# Autodesk Inventor assembly: s-assyypanel
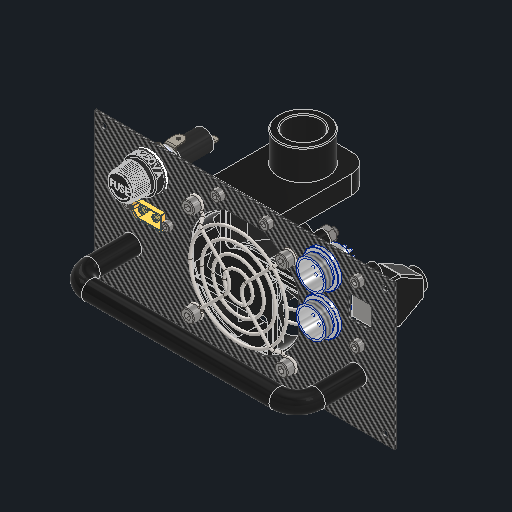
[picture p0: Inventor's stored thumbnail of the model, 512x512]
Saved by Autodesk Inventor 2022 (Build 260153000, 153)
## iProperties
Created: 2021-07-22
Part Number: s-assyypanel
Document SubType Name: Assembly
Designer: yuta0
Author: yuta0
## Documents named in this file (16)
- C:\Users\yuta0\Documents\GitHub\catchrobo_hardware\assy-scara\s-assyypanel.iam
- C:\Users\yuta0\Documents\GitHub\catchrobo_hardware\assy-scara\carbon_plate8.ipt
- C:\Users\yuta0\Documents\GitHub\catchrobo_hardware\assy-scara\Fan_Assembly.iam
- C:\Users\yuta0\Documents\GitHub\catchrobo_hardware\assy-scara\Fan protection grill 55023 - 60mm X 60mm.ipt
- C:\Users\yuta0\Documents\GitHub\catchrobo_hardware\assy-scara\SF372 10A 250VAC Fuse Holder.iam
- C:\Users\yuta0\Documents\GitHub\catchrobo_hardware\assy-scara\base11.ipt
- C:\Users\yuta0\Documents\GitHub\catchrobo_hardware\assy-scara\XT60E-M_V1.1.ipt
- C:\Users\yuta0\Documents\GitHub\catchrobo_hardware\assy-scara\UWANK10-120-27.ipt
- C:\Users\yuta0\Documents\GitHub\catchrobo_hardware\assy-scara\SB-305060.ipt
- C:\Users\yuta0\Documents\GitHub\catchrobo_hardware\assy-scara\CB3-5.ipt
- C:\Users\yuta0\Documents\GitHub\catchrobo_hardware\assy-scara\CB4-25.ipt
- C:\Users\yuta0\Documents\GitHub\catchrobo_hardware\assy-scara\LBNR4.ipt
- C:\Users\yuta0\Documents\GitHub\catchrobo_hardware\assy-scara\PLT-164-R-R.ipt
- C:\Users\yuta0\Documents\GitHub\catchrobo_hardware\assy-scara\USB2-MBMPAF-XXE.ipt
- C:\Users\yuta0\Documents\GitHub\catchrobo_hardware\assy-scara\CB2_5-6.ipt
- C:\Users\yuta0\Documents\GitHub\catchrobo_hardware\assy-scara\PLT-166-R-R.ipt
## Components (27 placed, 15 different names)
1. carbon_plate8:1 — メイト:10, メイト:12, メイト:13, メイト:14, メイト:15, 正接:1, メイト:21, メイト:22, 角度:2, メイト:27, メイト:28, メイト:30, メイト:31, メイト:32, メイト:33, メイト:34, メイト:35, メイト:40, メイト:41, メイト:42, メイト:43, メイト:44, メイト:46, メイト:47, メイト:48, メイト:49, メイト:50, メイト:51, メイト:54, メイト:55, メイト:56
2. PLT-164-R-R:1 — メイト:10, メイト:12, 角度:2
3. Fan_Assembly:1 [sub-assembly] — メイト:13, メイト:14, メイト:15, フラッシュ:1, メイト:16, メイト:25, メイト:26, 正接:2, メイト:29
4. Fan protection grill 55023 - 60mm X 60mm:1 — フラッシュ:1, メイト:16, 正接:1, 正接:3
5. SF372 10A 250VAC Fuse Holder:1 [sub-assembly] — メイト:21, メイト:22, 角度:1
6. Fan protection grill 55023 - 60mm X 60mm:2 — メイト:25, メイト:26, 正接:2, 正接:4
7. base11:1 — メイト:27, メイト:28, メイト:29, メイト:36, メイト:37, メイト:38, メイト:39
8. XT60E-M_V1.1:1 — メイト:30, メイト:31, メイト:32
9. UWANK10-120-27:1 — メイト:33, メイト:34, メイト:35
10. SB-305060:1 — メイト:36, メイト:39
11. SB-305060:2 — メイト:37, メイト:38
12. CB3-5:1 — メイト:42, メイト:43, メイト:53
13. CB3-5:2 — メイト:40, メイト:41, メイト:52
14. CB3-5:3 — メイト:46, メイト:47
15. CB3-5:4 — メイト:48, メイト:49
16. USB2-MBMPAF-XXE:1 — メイト:52, メイト:53, メイト:54
17. PLT-166-R-R:1 — メイト:55, メイト:56
18. CB4-25:1 — メイト:44, 正接:3, メイト:45
19. LBNR4:1 — メイト:45, 正接:4
20. CB4-25:2
21. LBNR4:2
22. CB4-25:3
23. LBNR4:3
24. CB4-25:4
25. LBNR4:4
26. CB2_5-6:1 — メイト:50, メイト:51
27. CB2_5-6:2
## Component patterns: (4 elements, first: CB4-25:1 + LBNR4:1), (2 elements, first: CB2_5-6:1)
## Relationships (47: Mate 40, Tangent 4, Angle 2, Flush 1)
- メイト:10 [Mate]: carbon_plate8:1 ↔ PLT-164-R-R:1
- メイト:12 [Mate]: carbon_plate8:1 ↔ PLT-164-R-R:1
- メイト:13 [Mate]: carbon_plate8:1 ↔ Fan_Assembly:1
- メイト:14 [Mate]: carbon_plate8:1 ↔ Fan_Assembly:1
- メイト:15 [Mate]: carbon_plate8:1 ↔ Fan_Assembly:1
- フラッシュ:1 [Flush]: Fan_Assembly:1 ↔ Fan protection grill 55023 - 60mm X 60mm:1
- メイト:16 [Mate]: Fan_Assembly:1 ↔ Fan protection grill 55023 - 60mm X 60mm:1
- 正接:1 [Tangent]: carbon_plate8:1 ↔ Fan protection grill 55023 - 60mm X 60mm:1
- メイト:21 [Mate]: carbon_plate8:1 ↔ SF372 10A 250VAC Fuse Holder:1
- メイト:22 [Mate]: carbon_plate8:1 ↔ SF372 10A 250VAC Fuse Holder:1
- 角度:1 [Angle] (0 deg): SF372 10A 250VAC Fuse Holder:1
- 角度:2 [Angle] (180 deg): carbon_plate8:1 ↔ PLT-164-R-R:1
- メイト:25 [Mate]: Fan_Assembly:1 ↔ Fan protection grill 55023 - 60mm X 60mm:2
- メイト:26 [Mate]: Fan_Assembly:1 ↔ Fan protection grill 55023 - 60mm X 60mm:2
- 正接:2 [Tangent]: Fan_Assembly:1 ↔ Fan protection grill 55023 - 60mm X 60mm:2
- メイト:27 [Mate]: carbon_plate8:1 ↔ base11:1
- メイト:28 [Mate]: carbon_plate8:1 ↔ base11:1
- メイト:29 [Mate]: Fan_Assembly:1 ↔ base11:1
- メイト:30 [Mate]: carbon_plate8:1 ↔ XT60E-M_V1.1:1
- メイト:31 [Mate]: carbon_plate8:1 ↔ XT60E-M_V1.1:1
- メイト:32 [Mate]: carbon_plate8:1 ↔ XT60E-M_V1.1:1
- メイト:33 [Mate]: carbon_plate8:1 ↔ UWANK10-120-27:1
- メイト:34 [Mate]: carbon_plate8:1 ↔ UWANK10-120-27:1
- メイト:35 [Mate]: carbon_plate8:1 ↔ UWANK10-120-27:1
- メイト:36 [Mate]: base11:1 ↔ SB-305060:1
- メイト:37 [Mate]: base11:1 ↔ SB-305060:2
- メイト:38 [Mate]: base11:1 ↔ SB-305060:2
- メイト:39 [Mate]: base11:1 ↔ SB-305060:1
- メイト:40 [Mate]: carbon_plate8:1 ↔ CB3-5:2
- メイト:41 [Mate]: carbon_plate8:1 ↔ CB3-5:2
- メイト:42 [Mate]: carbon_plate8:1 ↔ CB3-5:1
- メイト:43 [Mate]: carbon_plate8:1 ↔ CB3-5:1
- メイト:44 [Mate]: carbon_plate8:1 ↔ CB4-25:1
- 正接:3 [Tangent]: Fan protection grill 55023 - 60mm X 60mm:1 ↔ CB4-25:1
- メイト:45 [Mate]: CB4-25:1 ↔ LBNR4:1
- 正接:4 [Tangent]: Fan protection grill 55023 - 60mm X 60mm:2 ↔ LBNR4:1
- メイト:46 [Mate]: carbon_plate8:1 ↔ CB3-5:3
- メイト:47 [Mate]: carbon_plate8:1 ↔ CB3-5:3
- メイト:48 [Mate]: carbon_plate8:1 ↔ CB3-5:4
- メイト:49 [Mate]: carbon_plate8:1 ↔ CB3-5:4
- メイト:50 [Mate]: carbon_plate8:1 ↔ CB2_5-6:1
- メイト:51 [Mate]: carbon_plate8:1 ↔ CB2_5-6:1
- メイト:52 [Mate]: CB3-5:2 ↔ USB2-MBMPAF-XXE:1
- メイト:53 [Mate]: CB3-5:1 ↔ USB2-MBMPAF-XXE:1
- メイト:54 [Mate]: carbon_plate8:1 ↔ USB2-MBMPAF-XXE:1
- メイト:55 [Mate]: carbon_plate8:1 ↔ PLT-166-R-R:1
- メイト:56 [Mate]: carbon_plate8:1 ↔ PLT-166-R-R:1
